# Autodesk Inventor assembly: CathodeCage
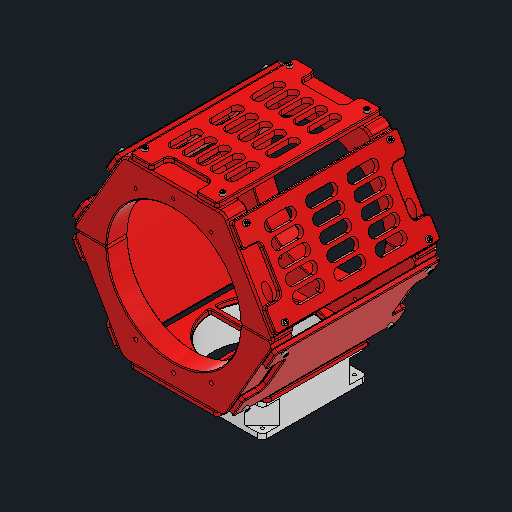
[picture p0: Inventor's stored thumbnail of the model, 512x512]
Saved by Autodesk Inventor 2026 (Build 300175050, 175E)
## iProperties
Created: 2023-12-04
Part Number: CathodeCage
Document SubType Name: Assembly
Designer: kuzmin
Author: kuzmin
## Documents named in this file (11)
- C:\Users\queezz\Dropbox\Drawings\PIHTI\Plasma Vessel\Cathode-Flange-Cage\CathodeCage.iam
- C:\Users\queezz\Dropbox\Drawings\PIHTI\Plasma Vessel\Cathode-Flange-Cage\Baseplate-for-ICF152-flange-outer-part.ipt
- C:\Users\queezz\Dropbox\Drawings\PIHTI\Plasma Vessel\Cathode-Flange-Cage\Cathode-Cover-Plate.ipt
- C:\Users\queezz\Dropbox\Drawings\PIHTI\Plasma Vessel\Cathode-Flange-Cage\AC-fan-case.ipt
- C:\Users\queezz\Dropbox\Drawings\PIHTI\Plasma Vessel\Cathode-Flange-Cage\Cathode-Cover-Plate-top-side-front.ipt
- C:\Users\queezz\Dropbox\Drawings\PIHTI\Plasma Vessel\Cathode-Flange-Cage\Cathode-Cover-Plate-bottom-side.ipt
- C:\Users\queezz\Dropbox\Drawings\PIHTI\Plasma Vessel\Cathode-Flange-Cage\Baseplate-for-ICF152-flange-outer-part-bottom.ipt
- C:\Users\queezz\Dropbox\Drawings\PIHTI\ContentCenter\Fastners\M4-nut.ipt
- C:\Users\queezz\Dropbox\Drawings\PIHTI\ContentCenter\Fastners\M4x30-SHCS.ipt
- C:\Users\queezz\Dropbox\Drawings\PIHTI\ContentCenter\Fastners\M3x10-SHCS.ipt
- C:\Users\queezz\Dropbox\Drawings\PIHTI\ContentCenter\Fastners\brass-insert-m3x5.ipt
## Components (57 placed, 10 different names)
1. Baseplate-for-ICF152-flange-outer-part:1 — Mate:5, Mate:6, Mate:7, Mate:13, Mate:14, Mate:22, Mate:23, Mate:38, Rotational:4, Rotational:5, Rigid:10, Rigid:40
2. Baseplate-for-ICF152-flange-outer-part:3 — Mate:3, Mate:4, Mate:8, Mate:21, Mate:24, Rotational:6, Rotational:7
3. Cathode-Cover-Plate:1 — Mate:28, Mate:29, Mate:30, Mate:32, Mate:35, Rotational:24, Rotational:25, Rotational:26, Rotational:27, Mate:39
4. AC-fan-case:1 — Mate:28, Mate:29, Mate:30
5. Cathode-Cover-Plate-top-side-front:1 — Mate:13, Mate:21, Mate:22, Rotational:12, Rotational:13, Rotational:14, Rotational:15
6. Cathode-Cover-Plate-top-side-front:2 — Mate:14, Mate:23, Mate:24, Rotational:16, Rotational:17, Rotational:18, Rotational:19
7. Cathode-Cover-Plate-top-side-front:3 — Mate:3, Mate:4, Mate:5, Mate:6, Mate:7, Mate:8, Rotational:8, Rotational:9, Rotational:10, Rotational:11
8. Cathode-Cover-Plate-bottom-side:1 — Rotational:28, Rotational:29, Rotational:30, Rotational:31, Rigid:50
9. Cathode-Cover-Plate-bottom-side:2 — Rotational:20, Rotational:21, Rotational:22, Rotational:23, Rigid:45
10. Baseplate-for-ICF152-flange-outer-part-bottom:1 — Mate:32, Mate:39, Mate:42, Rotational:34, Rotational:35, Rigid:43, Rigid:44, Rigid:46, Rigid:47, Rotational:38, Rigid:51
11. Baseplate-for-ICF152-flange-outer-part-bottom:2 — Mate:35, Mate:38, Mate:40, Mate:41, Mate:44, Rigid:6, Rigid:7, Rigid:39, Rigid:40, Rigid:41, Rigid:42, Rigid:45, Rigid:48, Rotational:36, Rigid:49, Rigid:50
12. JIS B 1176 - Metric M3 x 10:1 — Rotational:22
13. JIS B 1176 - Metric M3 x 10:2 — Rotational:21, Mate:44
14. JIS B 1176 - Metric M3 x 10:3 — Rotational:20
15. JIS B 1176 - Metric M3 x 10:4 — Rotational:8
16. JIS B 1176 - Metric M3 x 10:5 — Rotational:27
17. JIS B 1176 - Metric M3 x 10:6 — Rotational:26, Mate:40
18. JIS B 1176 - Metric M3 x 10:7 — Rotational:25
19. JIS B 1176 - Metric M3 x 10:8 — Rotational:24
20. JIS B 1176 - Metric M3 x 10:9 — Rotational:28, Mate:41
21. JIS B 1176 - Metric M3 x 10:10 — Rotational:29
22. JIS B 1176 - Metric M3 x 10:11 — Rotational:30, Mate:42
23. JIS B 1176 - Metric M3 x 10:12 — Rotational:31
24. JIS B 1176 - Metric M3 x 10:13 — Rotational:14
25. JIS B 1176 - Metric M3 x 10:14 — Rotational:15
26. JIS B 1176 - Metric M3 x 10:15 — Rotational:23
27. JIS B 1176 - Metric M3 x 10:16 — Rotational:13
28. JIS B 1176 - Metric M3 x 10:17 — Rotational:9
29. JIS B 1176 - Metric M3 x 10:18 — Rotational:10
30. JIS B 1176 - Metric M3 x 10:19 — Rotational:11
31. JIS B 1176 - Metric M3 x 10:20 — Rotational:12
32. JIS B 1176 - Metric M3 x 10:21 — Rotational:16
33. JIS B 1176 - Metric M3 x 10:22 — Rotational:17
34. JIS B 1176 - Metric M3 x 10:23 — Rotational:18
35. JIS B 1176 - Metric M3 x 10:24 — Rotational:19
36. JIS B 1181 -finished Class 1 - Metric Class 1 -finishedM4:1
37. JIS B 1181 -finished Class 1 - Metric Class 1 -finishedM4:2 — Rotational:38
38. JIS B 1181 -finished Class 1 - Metric Class 1 -finishedM4:3 — Rigid:49
39. JIS B 1181 -finished Class 1 - Metric Class 1 -finishedM4:4 — Rigid:51
40. JIS B 1176 - Metric M4 x 30:1 — Rotational:7
41. JIS B 1176 - Metric M4 x 30:2 — Rotational:6
42. JIS B 1176 - Metric M4 x 30:3 — Rotational:5
43. JIS B 1176 - Metric M4 x 30:4 — Rotational:4
44. brass-insert-m3x5:1 — Rigid:46
45. brass-insert-m3x5:2 — Rigid:47
46. brass-insert-m3x5:3 — Rotational:35
47. brass-insert-m3x5:4 — Rotational:34
48. brass-insert-m3x5:5 — Rigid:44
49. brass-insert-m3x5:6 — Rigid:43
50. brass-insert-m3x5:7 — Rigid:42
51. brass-insert-m3x5:8 — Rigid:6
52. brass-insert-m3x5:9 — Rigid:41
53. brass-insert-m3x5:10 — Rigid:7
54. brass-insert-m3x5:11 — Rotational:36
55. brass-insert-m3x5:12 — Rigid:48
56. brass-insert-m3x5:13 — Rigid:10
57. brass-insert-m3x5:14 — Rigid:39
## Relationships (71: RevoluteJoint 32, Mate 23, WeldJoint 16)
- Mate:3: Baseplate-for-ICF152-flange-outer-part:3 ↔ Cathode-Cover-Plate-top-side-front:3
- Mate:4: Baseplate-for-ICF152-flange-outer-part:3 ↔ Cathode-Cover-Plate-top-side-front:3
- Mate:5: Baseplate-for-ICF152-flange-outer-part:1 ↔ Cathode-Cover-Plate-top-side-front:3
- Mate:6: Baseplate-for-ICF152-flange-outer-part:1 ↔ Cathode-Cover-Plate-top-side-front:3
- Mate:7: Baseplate-for-ICF152-flange-outer-part:1 ↔ Cathode-Cover-Plate-top-side-front:3
- Mate:8: Baseplate-for-ICF152-flange-outer-part:3 ↔ Cathode-Cover-Plate-top-side-front:3
- Mate:13: Baseplate-for-ICF152-flange-outer-part:1 ↔ Cathode-Cover-Plate-top-side-front:1
- Mate:14: Baseplate-for-ICF152-flange-outer-part:1 ↔ Cathode-Cover-Plate-top-side-front:2
- Mate:21: Baseplate-for-ICF152-flange-outer-part:3 ↔ Cathode-Cover-Plate-top-side-front:1
- Mate:22: Baseplate-for-ICF152-flange-outer-part:1 ↔ Cathode-Cover-Plate-top-side-front:1
- Mate:23: Baseplate-for-ICF152-flange-outer-part:1 ↔ Cathode-Cover-Plate-top-side-front:2
- Mate:24: Baseplate-for-ICF152-flange-outer-part:3 ↔ Cathode-Cover-Plate-top-side-front:2
- Mate:28: Cathode-Cover-Plate:1 ↔ AC-fan-case:1
- Mate:29: Cathode-Cover-Plate:1 ↔ AC-fan-case:1
- Mate:30 (-101 mm): Cathode-Cover-Plate:1 ↔ AC-fan-case:1
- Mate:32: Cathode-Cover-Plate:1 ↔ Baseplate-for-ICF152-flange-outer-part-bottom:1
- Mate:35: Cathode-Cover-Plate:1 ↔ Baseplate-for-ICF152-flange-outer-part-bottom:2
- Mate:38: Baseplate-for-ICF152-flange-outer-part:1 ↔ Baseplate-for-ICF152-flange-outer-part-bottom:2
- Rotational:4 [RevoluteJoint]: Baseplate-for-ICF152-flange-outer-part:1 ↔ JIS B 1176 - Metric M4 x 30:4
- Rotational:5 [RevoluteJoint]: Baseplate-for-ICF152-flange-outer-part:1 ↔ JIS B 1176 - Metric M4 x 30:3
- Rotational:6 [RevoluteJoint]: Baseplate-for-ICF152-flange-outer-part:3 ↔ JIS B 1176 - Metric M4 x 30:2
- Rotational:7 [RevoluteJoint]: Baseplate-for-ICF152-flange-outer-part:3 ↔ JIS B 1176 - Metric M4 x 30:1
- Rotational:8 [RevoluteJoint]: Cathode-Cover-Plate-top-side-front:3 ↔ JIS B 1176 - Metric M3 x 10:4
- Rotational:9 [RevoluteJoint]: Cathode-Cover-Plate-top-side-front:3 ↔ JIS B 1176 - Metric M3 x 10:17
- Rotational:10 [RevoluteJoint]: Cathode-Cover-Plate-top-side-front:3 ↔ JIS B 1176 - Metric M3 x 10:18
- Rotational:11 [RevoluteJoint]: Cathode-Cover-Plate-top-side-front:3 ↔ JIS B 1176 - Metric M3 x 10:19
- Rotational:12 [RevoluteJoint]: Cathode-Cover-Plate-top-side-front:1 ↔ JIS B 1176 - Metric M3 x 10:20
- Rotational:13 [RevoluteJoint]: Cathode-Cover-Plate-top-side-front:1 ↔ JIS B 1176 - Metric M3 x 10:16
- Rotational:14 [RevoluteJoint]: Cathode-Cover-Plate-top-side-front:1 ↔ JIS B 1176 - Metric M3 x 10:13
- Rotational:15 [RevoluteJoint]: Cathode-Cover-Plate-top-side-front:1 ↔ JIS B 1176 - Metric M3 x 10:14
- Rotational:16 [RevoluteJoint]: Cathode-Cover-Plate-top-side-front:2 ↔ JIS B 1176 - Metric M3 x 10:21
- Rotational:17 [RevoluteJoint]: Cathode-Cover-Plate-top-side-front:2 ↔ JIS B 1176 - Metric M3 x 10:22
- Rotational:18 [RevoluteJoint]: Cathode-Cover-Plate-top-side-front:2 ↔ JIS B 1176 - Metric M3 x 10:23
- Rotational:19 [RevoluteJoint]: Cathode-Cover-Plate-top-side-front:2 ↔ JIS B 1176 - Metric M3 x 10:24
- Rotational:20 [RevoluteJoint]: Cathode-Cover-Plate-bottom-side:2 ↔ JIS B 1176 - Metric M3 x 10:3
- Rotational:21 [RevoluteJoint]: Cathode-Cover-Plate-bottom-side:2 ↔ JIS B 1176 - Metric M3 x 10:2
- Rotational:22 [RevoluteJoint]: Cathode-Cover-Plate-bottom-side:2 ↔ JIS B 1176 - Metric M3 x 10:1
- Rotational:23 [RevoluteJoint]: Cathode-Cover-Plate-bottom-side:2 ↔ JIS B 1176 - Metric M3 x 10:15
- Rotational:24 [RevoluteJoint]: Cathode-Cover-Plate:1 ↔ JIS B 1176 - Metric M3 x 10:8
- Rotational:25 [RevoluteJoint]: Cathode-Cover-Plate:1 ↔ JIS B 1176 - Metric M3 x 10:7
- Rotational:26 [RevoluteJoint]: Cathode-Cover-Plate:1 ↔ JIS B 1176 - Metric M3 x 10:6
- Rotational:27 [RevoluteJoint]: Cathode-Cover-Plate:1 ↔ JIS B 1176 - Metric M3 x 10:5
- Rotational:28 [RevoluteJoint]: Cathode-Cover-Plate-bottom-side:1 ↔ JIS B 1176 - Metric M3 x 10:9
- Rotational:29 [RevoluteJoint]: Cathode-Cover-Plate-bottom-side:1 ↔ JIS B 1176 - Metric M3 x 10:10
- Rotational:30 [RevoluteJoint]: Cathode-Cover-Plate-bottom-side:1 ↔ JIS B 1176 - Metric M3 x 10:11
- Rotational:31 [RevoluteJoint]: Cathode-Cover-Plate-bottom-side:1 ↔ JIS B 1176 - Metric M3 x 10:12
- Mate:39: Cathode-Cover-Plate:1 ↔ Baseplate-for-ICF152-flange-outer-part-bottom:1
- Mate:40: Baseplate-for-ICF152-flange-outer-part-bottom:2 ↔ JIS B 1176 - Metric M3 x 10:6
- Mate:41: Baseplate-for-ICF152-flange-outer-part-bottom:2 ↔ JIS B 1176 - Metric M3 x 10:9
- Mate:42: Baseplate-for-ICF152-flange-outer-part-bottom:1 ↔ JIS B 1176 - Metric M3 x 10:11
- Mate:44: Baseplate-for-ICF152-flange-outer-part-bottom:2 ↔ JIS B 1176 - Metric M3 x 10:2
- Rigid:6 [WeldJoint]: Baseplate-for-ICF152-flange-outer-part-bottom:2 ↔ brass-insert-m3x5:8
- Rigid:7 [WeldJoint]: Baseplate-for-ICF152-flange-outer-part-bottom:2 ↔ brass-insert-m3x5:10
- Rotational:34 [RevoluteJoint]: Baseplate-for-ICF152-flange-outer-part-bottom:1 ↔ brass-insert-m3x5:4
- Rotational:35 [RevoluteJoint]: Baseplate-for-ICF152-flange-outer-part-bottom:1 ↔ brass-insert-m3x5:3
- Rigid:39 [WeldJoint]: Baseplate-for-ICF152-flange-outer-part-bottom:2 ↔ brass-insert-m3x5:14
- Rigid:10 [WeldJoint]: Baseplate-for-ICF152-flange-outer-part:1 ↔ brass-insert-m3x5:13
- Rigid:40 [WeldJoint]: Baseplate-for-ICF152-flange-outer-part:1 ↔ Baseplate-for-ICF152-flange-outer-part-bottom:2
- Rigid:41 [WeldJoint]: Baseplate-for-ICF152-flange-outer-part-bottom:2 ↔ brass-insert-m3x5:9
- Rigid:42 [WeldJoint]: Baseplate-for-ICF152-flange-outer-part-bottom:2 ↔ brass-insert-m3x5:7
- Rigid:43 [WeldJoint]: Baseplate-for-ICF152-flange-outer-part-bottom:1 ↔ brass-insert-m3x5:6
- Rigid:44 [WeldJoint]: Baseplate-for-ICF152-flange-outer-part-bottom:1 ↔ brass-insert-m3x5:5
- Rigid:45 [WeldJoint]: Cathode-Cover-Plate-bottom-side:2 ↔ Baseplate-for-ICF152-flange-outer-part-bottom:2
- Rigid:46 [WeldJoint]: Baseplate-for-ICF152-flange-outer-part-bottom:1 ↔ brass-insert-m3x5:1
- Rigid:47 [WeldJoint]: Baseplate-for-ICF152-flange-outer-part-bottom:1 ↔ brass-insert-m3x5:2
- Rigid:48 [WeldJoint]: Baseplate-for-ICF152-flange-outer-part-bottom:2 ↔ brass-insert-m3x5:12
- Rotational:36 [RevoluteJoint]: Baseplate-for-ICF152-flange-outer-part-bottom:2 ↔ brass-insert-m3x5:11
- Rigid:49 [WeldJoint]: Baseplate-for-ICF152-flange-outer-part-bottom:2 ↔ JIS B 1181 -finished Class 1 - Metric Class 1 -finishedM4:3
- Rotational:38 [RevoluteJoint]: Baseplate-for-ICF152-flange-outer-part-bottom:1 ↔ JIS B 1181 -finished Class 1 - Metric Class 1 -finishedM4:2
- Rigid:50 [WeldJoint]: Cathode-Cover-Plate-bottom-side:1 ↔ Baseplate-for-ICF152-flange-outer-part-bottom:2
- Rigid:51 [WeldJoint]: Baseplate-for-ICF152-flange-outer-part-bottom:1 ↔ JIS B 1181 -finished Class 1 - Metric Class 1 -finishedM4:4
